# Autodesk Inventor assembly: axis
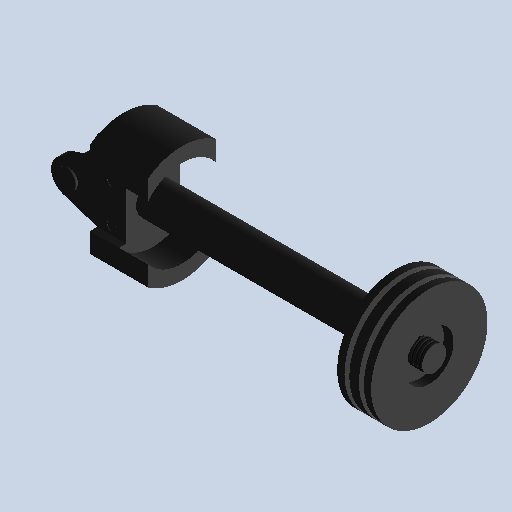
[picture p0: Inventor's stored thumbnail of the model, 512x512]
Saved by Autodesk Inventor 2025.1 (Build 291241000, 241)
## iProperties
Created: 2024-09-18
Part Number: axis
Document SubType Name: Assembly
Designer: ffogue
Author: ffogue
## Documents named in this file (8)
- C:\Users\ffogue\Documents\Inventor\Cylinder Radial Steam Engine\axis.iam
- C:\Users\ffogue\Documents\Inventor\Cylinder Radial Steam Engine\41.ipt
- C:\Users\ffogue\Documents\Inventor\Cylinder Radial Steam Engine\40.ipt
- C:\Users\ffogue\Documents\Inventor\Cylinder Radial Steam Engine\42.ipt
- C:\Users\ffogue\Documents\Inventor\Cylinder Radial Steam Engine\43.ipt
- C:\Users\ffogue\Documents\Inventor\Cylinder Radial Steam Engine\43A.ipt
- C:\Users\ffogue\Documents\Inventor\Cylinder Radial Steam Engine\44.ipt
- C:\Users\ffogue\Documents\Inventor\Cylinder Radial Steam Engine\52.ipt
## Components (10 placed, 7 different names)
1. 41:1 — Mate:1, Mate:2, Insert:1, Mate:3, Insert:2
2. 40:1 — Mate:1, Mate:2, Insert:1, Mate:9, Insert:8, Mate:10, Insert:9
3. 42:1 — Mate:3, Insert:2, Mate:4, Mate:5, Insert:3, Insert:4
4. 43:1 — Mate:5, Insert:3
5. 43:2 — Mate:4, Insert:4, Mate:6, Insert:5, Mate:7, Mate:8, Insert:6, Insert:7
6. 43A:1 — Mate:6, Insert:5
7. 44:2 — Mate:8, Insert:6
8. 44:3 — Mate:7, Insert:7
9. 52:1 — Mate:9, Insert:8
10. 52:2 — Mate:10, Insert:9
## Relationships (19: Mate 10, Insert 9)
- Mate:1: 41:1 ↔ 40:1
- Mate:2: 41:1 ↔ 40:1
- Insert:1: 41:1 ↔ 40:1
- Mate:3: 41:1 ↔ 42:1
- Insert:2: 41:1 ↔ 42:1
- Mate:4: 42:1 ↔ 43:2
- Mate:5: 42:1 ↔ 43:1
- Insert:3: 42:1 ↔ 43:1
- Insert:4: 42:1 ↔ 43:2
- Mate:6: 43:2 ↔ 43A:1
- Insert:5 (-11.5 mm): 43:2 ↔ 43A:1
- Mate:7: 43:2 ↔ 44:3
- Mate:8: 43:2 ↔ 44:2
- Insert:6 (-11 mm): 43:2 ↔ 44:2
- Insert:7 (-11 mm): 43:2 ↔ 44:3
- Mate:9: 40:1 ↔ 52:1
- Insert:8: 40:1 ↔ 52:1
- Mate:10: 40:1 ↔ 52:2
- Insert:9: 40:1 ↔ 52:2
